# Autodesk Inventor assembly: Assembly2
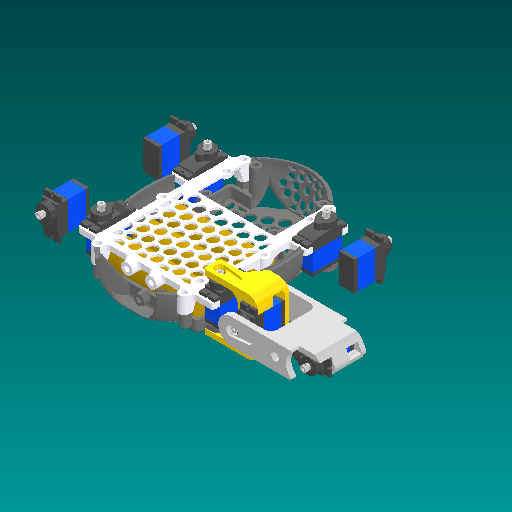
[picture p0: Inventor's stored thumbnail of the model, 512x512]
Saved by Autodesk Inventor 2026 (Build 300175050, 175E)
## iProperties
Created: 2026-02-15
Part Number: Assembly2
Document SubType Name: Assembly
Designer: Gir
Author: Gir
## Documents named in this file (3)
- F:\Documentos\Jota\jRobot\Robots\Quad Bot Jota\Modelos 3D Jota QuadBot\Assembly2.iam
- F:\Documentos\Jota\jRobot\Robots\Quad Bot Jota\Modelos 3D Jota QuadBot\body_d_L_Screws.ipt
- F:\Documentos\Jota\jRobot\Maquetas\towerpro-mg92b-1.snapshot.20\TowerPro_MG92B\TowerPro_MG92B\TowerPro_MG92B\TowerPro_MG92B.iam
## Components (10 placed, 2 different names)
1. body_d_L_Screws:1 — Insert:1, Insert:2, Insert:3, Insert:4, Insert:5, Insert:6, Insert:7, Insert:8, Insert:9, Insert:10, Insert:11, Insert:12, Insert:13, Insert:14, Insert:15, Insert:16, Insert:17, Insert:18
2. TowerPro_MG92B:1 [sub-assembly] — Insert:3, Insert:4
3. TowerPro_MG92B:2 [sub-assembly] — Insert:1, Insert:2
4. TowerPro_MG92B:3 [sub-assembly] — Insert:7, Insert:8
5. TowerPro_MG92B:4 [sub-assembly] — Insert:5, Insert:6
6. TowerPro_MG92B:5 [sub-assembly] — Insert:9, Insert:10
7. TowerPro_MG92B:6 [sub-assembly] — Insert:11, Insert:12
8. TowerPro_MG92B:7 [sub-assembly] — Insert:13, Insert:14
9. TowerPro_MG92B:8 [sub-assembly] — Insert:15, Insert:16
10. TowerPro_MG92B:9 [sub-assembly] — Insert:17, Insert:18
## Relationships (18: Insert 18)
- Insert:1: body_d_L_Screws:1 ↔ TowerPro_MG92B:2
- Insert:2: body_d_L_Screws:1 ↔ TowerPro_MG92B:2
- Insert:3: body_d_L_Screws:1 ↔ TowerPro_MG92B:1
- Insert:4: body_d_L_Screws:1 ↔ TowerPro_MG92B:1
- Insert:5: body_d_L_Screws:1 ↔ TowerPro_MG92B:4
- Insert:6: body_d_L_Screws:1 ↔ TowerPro_MG92B:4
- Insert:7: body_d_L_Screws:1 ↔ TowerPro_MG92B:3
- Insert:8: body_d_L_Screws:1 ↔ TowerPro_MG92B:3
- Insert:9: body_d_L_Screws:1 ↔ TowerPro_MG92B:5
- Insert:10: body_d_L_Screws:1 ↔ TowerPro_MG92B:5
- Insert:11: body_d_L_Screws:1 ↔ TowerPro_MG92B:6
- Insert:12: body_d_L_Screws:1 ↔ TowerPro_MG92B:6
- Insert:13: body_d_L_Screws:1 ↔ TowerPro_MG92B:7
- Insert:14: body_d_L_Screws:1 ↔ TowerPro_MG92B:7
- Insert:15: body_d_L_Screws:1 ↔ TowerPro_MG92B:8
- Insert:16: body_d_L_Screws:1 ↔ TowerPro_MG92B:8
- Insert:17: body_d_L_Screws:1 ↔ TowerPro_MG92B:9
- Insert:18: body_d_L_Screws:1 ↔ TowerPro_MG92B:9
